# Autodesk Inventor assembly: Leg_Loadpipe_Connector
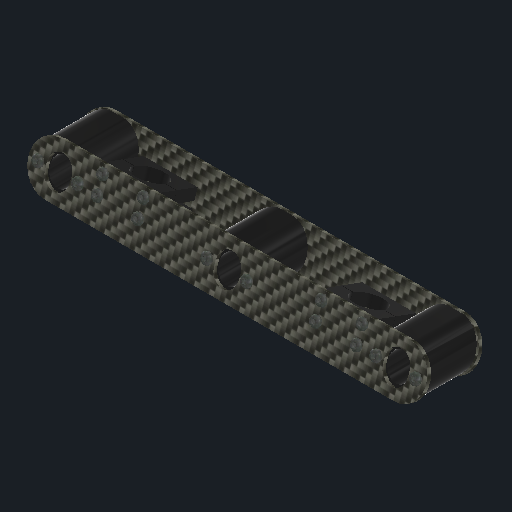
[picture p0: Inventor's stored thumbnail of the model, 512x512]
Saved by Autodesk Inventor 2025 (Build 290162010, 162A)
## iProperties
Created: 2023-12-05
Part Number: Leg_Loadpipe_Connector
Document SubType Name: Assembly
Designer: dzw04
Mass: 91.5441 g
Surface Area: 481.179 cm^2
Volume: 54.4026 cm^3
Density: 1.68272 g/cm^3
Author: dzw04
## Documents named in this file (4)
- C:\Users\dhrzw\OneDrive - Saxion\Sarax_Pack_And_Go\Workspaces\Workspace\SARAX\01. CAD\01. 3D_Drawing\02. Sub_Assemblies\Landing_Gear\02. Sub_Assemblies\Leg_Loadpipe_Connector.iam
- C:\Users\dhrzw\OneDrive - Saxion\Sarax_Pack_And_Go\Workspaces\Workspace\SARAX\01. CAD\01. 3D_Drawing\02. Sub_Assemblies\Landing_Gear\02. Sub_Assemblies\Leg_Loadpipe_Mount.iam
- C:\Users\dhrzw\OneDrive - Saxion\Sarax_Pack_And_Go\Workspaces\Workspace\SARAX\01. CAD\01. 3D_Drawing\02. Sub_Assemblies\Landing_Gear\02. Sub_Assemblies\16mm_Tube_Connector.iam
- C:\Users\dhrzw\OneDrive - Saxion\Sarax_Pack_And_Go\Workspaces\Workspace\SARAX\01. CAD\01. 3D_Drawing\02. Sub_Assemblies\Landing_Gear\01. Parts\Leg_Loadpipe_Plate.ipt
## Components (9 placed, 3 different names)
1. Leg_Loadpipe_Plate:1 — Mate:1, Mate:5, Mate:6, Mate:7, Mate:11, Mate:12, Mate:13, Mate:14, Mate:15, Mate:16, Mate:19, Mate:21, Mate:22, Mate:23, Mate:24, Mate:25
2. Leg_Loadpipe_Plate:2 — Mate:17, Mate:18, Mate:20, Mate:26, Mate:27, Mate:28, Mate:29, Mate:30, Mate:31, Mate:32, Mate:33
3. Leg_Loadpipe_Mount:1 [sub-assembly] — Mate:7, Mate:17, Mate:19
4. Leg_Loadpipe_Mount:2 [sub-assembly] — Mate:1, Mate:5, Mate:6
5. Leg_Loadpipe_Mount:3 [sub-assembly] — Mate:11, Mate:12, Mate:18, Mate:20, Mate:21
6. 16mm_Tube_Connector:1 [sub-assembly] — Mate:13, Mate:25, Mate:26, Mate:31
7. 16mm_Tube_Connector:2 [sub-assembly] — Mate:14, Mate:24, Mate:27, Mate:30
8. 16mm_Tube_Connector:3 [sub-assembly] — Mate:15, Mate:23, Mate:28, Mate:33
9. 16mm_Tube_Connector:4 [sub-assembly] — Mate:16, Mate:22, Mate:29, Mate:32
## Relationships (27: Mate 27)
- Mate:1: Leg_Loadpipe_Plate:1 ↔ Leg_Loadpipe_Mount:2
- Mate:5: Leg_Loadpipe_Plate:1 ↔ Leg_Loadpipe_Mount:2
- Mate:6: Leg_Loadpipe_Plate:1 ↔ Leg_Loadpipe_Mount:2
- Mate:7: Leg_Loadpipe_Plate:1 ↔ Leg_Loadpipe_Mount:1
- Mate:11: Leg_Loadpipe_Plate:1 ↔ Leg_Loadpipe_Mount:3
- Mate:12: Leg_Loadpipe_Plate:1 ↔ Leg_Loadpipe_Mount:3
- Mate:13: Leg_Loadpipe_Plate:1 ↔ 16mm_Tube_Connector:1
- Mate:14: Leg_Loadpipe_Plate:1 ↔ 16mm_Tube_Connector:2
- Mate:15: Leg_Loadpipe_Plate:1 ↔ 16mm_Tube_Connector:3
- Mate:16: Leg_Loadpipe_Plate:1 ↔ 16mm_Tube_Connector:4
- Mate:17: Leg_Loadpipe_Plate:2 ↔ Leg_Loadpipe_Mount:1
- Mate:18: Leg_Loadpipe_Plate:2 ↔ Leg_Loadpipe_Mount:3
- Mate:19: Leg_Loadpipe_Plate:1 ↔ Leg_Loadpipe_Mount:1
- Mate:20 (0.1 mm): Leg_Loadpipe_Plate:2 ↔ Leg_Loadpipe_Mount:3
- Mate:21: Leg_Loadpipe_Plate:1 ↔ Leg_Loadpipe_Mount:3
- Mate:22: Leg_Loadpipe_Plate:1 ↔ 16mm_Tube_Connector:4
- Mate:23: Leg_Loadpipe_Plate:1 ↔ 16mm_Tube_Connector:3
- Mate:24: Leg_Loadpipe_Plate:1 ↔ 16mm_Tube_Connector:2
- Mate:25: Leg_Loadpipe_Plate:1 ↔ 16mm_Tube_Connector:1
- Mate:26: Leg_Loadpipe_Plate:2 ↔ 16mm_Tube_Connector:1
- Mate:27: Leg_Loadpipe_Plate:2 ↔ 16mm_Tube_Connector:2
- Mate:28: Leg_Loadpipe_Plate:2 ↔ 16mm_Tube_Connector:3
- Mate:29: Leg_Loadpipe_Plate:2 ↔ 16mm_Tube_Connector:4
- Mate:30: Leg_Loadpipe_Plate:2 ↔ 16mm_Tube_Connector:2
- Mate:31: Leg_Loadpipe_Plate:2 ↔ 16mm_Tube_Connector:1
- Mate:32: Leg_Loadpipe_Plate:2 ↔ 16mm_Tube_Connector:4
- Mate:33: Leg_Loadpipe_Plate:2 ↔ 16mm_Tube_Connector:3
